# Autodesk Inventor assembly: ND.NeuroLink._Main
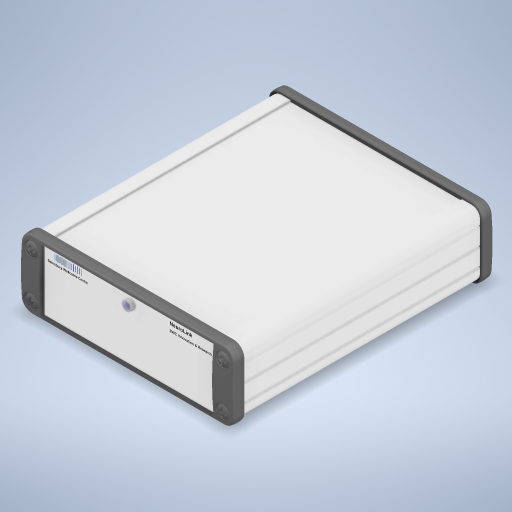
[picture p0: Inventor's stored thumbnail of the model, 512x512]
Saved by Autodesk Inventor 2023 (Build 270158000, 158)
## iProperties
Created: 2022-03-22
Part Number: ND.NeuroLink._Main
Document SubType Name: Assembly
Designer: Graeme
Author: Graeme
## Documents named in this file (7)
- C:\Work\Projects\swc_perturbation_treadmill\mCAD\Neural Link Box\ND.NeuroLink._Main.iam
- C:\Work\Projects\swc_perturbation_treadmill\mCAD\Neural Link Box\1457L1201EBK\1457L1201EBK.iam
- C:\Work\Projects\swc_perturbation_treadmill\mCAD\Neural Link Box\BaseBoard\BaseBoard.iam
- C:\Work\Projects\swc_perturbation_treadmill\mCAD\Neural Link Box\raspberry-pi-pico\Raspberry Pi Pico-R3.iam
- C:\Work\Projects\swc_perturbation_treadmill\mCAD\Neural Link Box\mentor_1216-1001-1\1216.1001.ipt
- C:\Work\Projects\swc_perturbation_treadmill\mCAD\Neural Link Box\mentor_1216-1001-1\1216.1001_head.iam
- C:\Work\Projects\swc_perturbation_treadmill\mCAD\Neural Link Box\mentor_1216-1001-1\1216.1001_LightPipe.ipt
## Components (6 placed, 6 different names)
1. 1457L1201EBK:1 [sub-assembly] — Mate:1, Mate:2, Flush:1, Mate:8, Mate:10
2. BaseBoard:1 [sub-assembly] — Mate:1, Mate:2, Flush:1, Mate:3, Mate:4, Flush:2, Mate:5, Mate:6, Mate:7
3. Raspberry Pi Pico-R3:1 [sub-assembly] — Mate:3, Mate:4, Flush:2
4. 1216.1001:1 — Mate:5, Mate:6, Mate:7
5. 1216.1001_head:1 [sub-assembly] — Mate:8, Mate:9, Mate:10
6. 1216.1001_LightPipe:1 — Flush:3
## Relationships (13: Mate 10, Flush 3)
- Mate:1: 1457L1201EBK:1 ↔ BaseBoard:1
- Mate:2: 1457L1201EBK:1 ↔ BaseBoard:1
- Flush:1 (1.3 mm): 1457L1201EBK:1 ↔ BaseBoard:1
- Mate:3: BaseBoard:1 ↔ Raspberry Pi Pico-R3:1
- Mate:4 (0.075 mm): BaseBoard:1 ↔ Raspberry Pi Pico-R3:1
- Flush:2: BaseBoard:1 ↔ Raspberry Pi Pico-R3:1
- Mate:5: BaseBoard:1 ↔ 1216.1001:1
- Mate:6: BaseBoard:1 ↔ 1216.1001:1
- Mate:7: BaseBoard:1 ↔ 1216.1001:1
- Mate:8: 1457L1201EBK:1 ↔ 1216.1001_head:1
- Mate:9: 1216.1001_head:1
- Mate:10 (2.2 mm): 1457L1201EBK:1 ↔ 1216.1001_head:1
- Flush:3: 1216.1001_LightPipe:1
